# Autodesk Inventor assembly: Assembly1
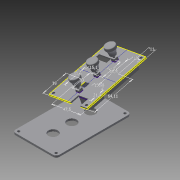
[picture p0: Inventor's stored thumbnail of the model, 180x180]
Saved by Autodesk Inventor 2013 (Build 170138000, 138)
## iProperties
Created: 2013-01-11
Part Number: Assembly1
Document SubType Name: Assembly
Designer: md
Author: md
## Documents named in this file (4)
- X:\Projects\hexasense\enclosure\sense_board\Assembly1.iam
- X:\Projects\hexasense\enclosure\sense_board\frontplatte.ipt
- X:\Projects\hexasense\enclosure\sense_board\pushbutton.ipt
- X:\Projects\hexasense\enclosure\sense_board\PCB-Model.ipt
## Components (5 placed, 3 different names)
1. frontplatte:1
2. pushbutton:1 — Insert:2
3. pushbutton:2 — Insert:3
4. pushbutton:3 — Insert:1
5. PCB-Model:1 — Insert:1, Insert:2, Insert:3
## Relationships (3: Insert 3)
- Insert:1 (-5 mm): pushbutton:3 ↔ PCB-Model:1
- Insert:2 (-5 mm): pushbutton:1 ↔ PCB-Model:1
- Insert:3 (-5 mm): pushbutton:2 ↔ PCB-Model:1
